# Autodesk Inventor assembly: Torso_automi
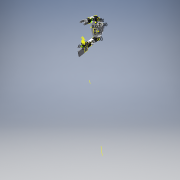
[picture p0: Inventor's stored thumbnail of the model, 180x180]
Saved by Autodesk Inventor 2018 (Build 220112000, 112)
## iProperties
Created: 2018-06-24
Part Number: Torso_automi
Document SubType Name: Assembly
Designer: ayush
Author: ayush
## Documents named in this file (12)
- C:\Users\Abhay\Desktop\Huro\gripper\Torso_automi.iam
- C:\Users\Abhay\Desktop\Huro\_18 Summers\Biped\AX-18A.iam
- C:\Users\Abhay\Desktop\Huro\_18 Summers\Biped\Chest_up.ipt
- C:\Users\Abhay\Desktop\Huro\_18 Summers\Biped\AX18_Frame.ipt
- C:\Users\Abhay\Desktop\Huro\_18 Summers\Biped\FR04_Ax18.ipt
- C:\Users\Abhay\Desktop\Huro\_18 Summers\Biped\Chest_mid.ipt
- C:\Users\Abhay\Desktop\Huro\_18 Summers\Biped\FP04_Ax18.ipt
- C:\Users\Abhay\Desktop\Huro\_18 Summers\Biped\AX18_2nd_Frame.ipt
- C:\Users\Abhay\Desktop\Huro\_18 Summers\Biped\FP04-F2.ipt
- C:\Users\Abhay\Desktop\Huro\_18 Summers\Biped\BPF-BU.ipt
- C:\Users\Abhay\Desktop\Huro\_18 Summers\Biped\BPF-WA.ipt
- C:\Users\Abhay\Desktop\Huro\gripper\Assembly1.iam
## Components (33 placed, 11 different names)
1. AX-18A:1 [sub-assembly] — Rigid:1, Rotational:3, Mate:3, Mate:5
2. Chest_up:1 — Rigid:1, Rotational:1, Mate:1
3. AX-18A:2 [sub-assembly] — Rotational:1, Mate:1, Rigid:2, Rotational:2, Mate:2, Mate:6
4. Chest_up:2 — Rigid:2
5. AX18_Frame:1 — Rotational:3, Mate:3
6. AX18_Frame:2 — Rotational:2, Mate:2, Rotational:9, Mate:9
7. AX-18A:5 [sub-assembly] — Rotational:6, Rotational:8, Mate:8, Rigid:23, Rotational:23
8. AX-18A:6 [sub-assembly] — Rotational:5, Rotational:7, Mate:7, Rigid:25, Rotational:25
9. FR04_Ax18:1 — Mate:5, Rotational:5
10. FR04_Ax18:2 — Mate:6, Rotational:6
11. AX18_Frame:3 — Rotational:7, Mate:7, Rotational:10, Mate:10
12. AX18_Frame:4 — Rotational:8, Mate:8, Rotational:11, Mate:11
13. Chest_mid:1 — Rotational:9, Mate:9, Rotational:20, Mate:16
14. FP04_Ax18:1 — Rotational:11, Mate:11, Rotational:12
15. FP04_Ax18:2 — Rotational:10, Mate:10, Rotational:13
16. AX-18A:7 [sub-assembly] — Rotational:12, Rotational:15, Mate:13, Rigid:24, Rotational:24
17. AX-18A:8 [sub-assembly] — Rotational:13, Rotational:14, Mate:12, Rotational:26, Rotational:27
18. AX18_Frame:5 — Rotational:14, Mate:12, Rotational:16, Mate:14
19. AX18_Frame:6 — Rotational:15, Mate:13, Rotational:28, Mate:18
20. FP04_Ax18:4 — Rotational:16, Mate:14
21. AX-18A:11 [sub-assembly] — Rotational:20, Mate:16, Rigid:22
22. AX18_2nd_Frame:1 — Rigid:22, Rotational:21, Mate:17
23. AX-18A:12 [sub-assembly] — Rotational:21, Mate:17, Rotational:22
24. FP04-F2:1 — Rotational:22
25. BPF-BU:1 — Rotational:26
26. BPF-BU:2 — Rigid:25
27. BPF-BU:3 — Rigid:23
28. BPF-BU:4 — Rigid:24
29. BPF-WA:1 — Rotational:25
30. BPF-WA:2 — Rotational:27
31. BPF-WA:3 — Rotational:24
32. BPF-WA:4 — Rotational:23
33. Assembly1:1 [sub-assembly] — Rotational:28, Mate:18
## Relationships (46: RevoluteJoint 24, Mate 16, WeldJoint 6)
- Rigid:1 [WeldJoint]: AX-18A:1 ↔ Chest_up:1
- Rotational:1 [RevoluteJoint]: Chest_up:1 ↔ AX-18A:2
- Mate:1: Chest_up:1 ↔ AX-18A:2
- Rigid:2 [WeldJoint]: AX-18A:2 ↔ Chest_up:2
- Rotational:2 [RevoluteJoint] (-1 mm): AX-18A:2 ↔ AX18_Frame:2
- Mate:2: AX-18A:2 ↔ AX18_Frame:2
- Rotational:3 [RevoluteJoint] (-1 mm): AX-18A:1 ↔ AX18_Frame:1
- Mate:3: AX-18A:1 ↔ AX18_Frame:1
- Mate:5: AX-18A:1 ↔ FR04_Ax18:1
- Mate:6: AX-18A:2 ↔ FR04_Ax18:2
- Rotational:5 [RevoluteJoint]: AX-18A:6 ↔ FR04_Ax18:1
- Rotational:6 [RevoluteJoint]: AX-18A:5 ↔ FR04_Ax18:2
- Rotational:7 [RevoluteJoint] (-1 mm): AX-18A:6 ↔ AX18_Frame:3
- Mate:7: AX-18A:6 ↔ AX18_Frame:3
- Rotational:8 [RevoluteJoint]: AX-18A:5 ↔ AX18_Frame:4
- Mate:8: AX-18A:5 ↔ AX18_Frame:4
- Rotational:9 [RevoluteJoint]: AX18_Frame:2 ↔ Chest_mid:1
- Mate:9: AX18_Frame:2 ↔ Chest_mid:1
- Rotational:10 [RevoluteJoint]: AX18_Frame:3 ↔ FP04_Ax18:2
- Mate:10: AX18_Frame:3 ↔ FP04_Ax18:2
- Rotational:11 [RevoluteJoint]: AX18_Frame:4 ↔ FP04_Ax18:1
- Mate:11: AX18_Frame:4 ↔ FP04_Ax18:1
- Rotational:12 [RevoluteJoint] (-1 mm): FP04_Ax18:1 ↔ AX-18A:7
- Rotational:13 [RevoluteJoint] (-1 mm): FP04_Ax18:2 ↔ AX-18A:8
- Rotational:14 [RevoluteJoint] (-1 mm): AX-18A:8 ↔ AX18_Frame:5
- Mate:12: AX-18A:8 ↔ AX18_Frame:5
- Rotational:15 [RevoluteJoint] (-1 mm): AX-18A:7 ↔ AX18_Frame:6
- Mate:13: AX-18A:7 ↔ AX18_Frame:6
- Rotational:16 [RevoluteJoint]: AX18_Frame:5 ↔ FP04_Ax18:4
- Mate:14: AX18_Frame:5 ↔ FP04_Ax18:4
- Rotational:20 [RevoluteJoint]: Chest_mid:1 ↔ AX-18A:11
- Mate:16: Chest_mid:1 ↔ AX-18A:11
- Rigid:22 [WeldJoint]: AX-18A:11 ↔ AX18_2nd_Frame:1
- Rotational:21 [RevoluteJoint]: AX18_2nd_Frame:1 ↔ AX-18A:12
- Mate:17: AX18_2nd_Frame:1 ↔ AX-18A:12
- Rotational:22 [RevoluteJoint]: AX-18A:12 ↔ FP04-F2:1
- Rigid:23 [WeldJoint]: AX-18A:5 ↔ BPF-BU:3
- Rotational:23 [RevoluteJoint]: AX-18A:5 ↔ BPF-WA:4
- Rigid:24 [WeldJoint]: AX-18A:7 ↔ BPF-BU:4
- Rotational:24 [RevoluteJoint]: AX-18A:7 ↔ BPF-WA:3
- Rigid:25 [WeldJoint]: AX-18A:6 ↔ BPF-BU:2
- Rotational:25 [RevoluteJoint]: AX-18A:6 ↔ BPF-WA:1
- Rotational:26 [RevoluteJoint]: AX-18A:8 ↔ BPF-BU:1
- Rotational:27 [RevoluteJoint]: AX-18A:8 ↔ BPF-WA:2
- Rotational:28 [RevoluteJoint]: AX18_Frame:6 ↔ Assembly1:1
- Mate:18: AX18_Frame:6 ↔ Assembly1:1
